# Autodesk Inventor assembly: capAndBase
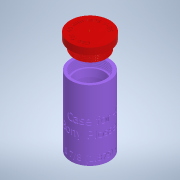
[picture p0: Inventor's stored thumbnail of the model, 180x180]
Saved by Autodesk Inventor 2021.1 (Build 251245010, 245A)
## iProperties
Created: 2020-10-23
Part Number: capAndBase
Document SubType Name: Assembly
Designer: robst
Author: robst
## Documents named in this file (3)
- C:\git\CAD-Development\robSteele\ShapeWays\TelescopeProjects\eyepieceCases\capAndBase.iam
- C:\git\CAD-Development\robSteele\ShapeWays\TelescopeProjects\eyepieceCases\BaseForSvBonyPlosse-40mm-V03.ipt
- C:\git\CAD-Development\robSteele\ShapeWays\TelescopeProjects\eyepieceCases\CapForSvBonyPlosse-40mm-V06.ipt
## Components (2 placed, 2 different names)
1. BaseForSvBonyPlosse-40mm-V03:1 — Insert:1
2. CapForSvBonyPlosse-40mm-V06:1 — Insert:1
## Relationships (1: Insert 1)
- Insert:1 (25.4 mm): BaseForSvBonyPlosse-40mm-V03:1 ↔ CapForSvBonyPlosse-40mm-V06:1
